# Autodesk Inventor assembly: TR1 Actuator
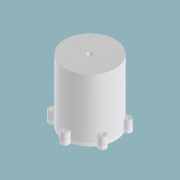
[picture p0: Inventor's stored thumbnail of the model, 180x180]
Saved by Autodesk Inventor 2017 SP1 (Build 210196100, 196)
## iProperties
Created: 2018-10-09
Part Number: TR1 Actuator
Document SubType Name: Assembly
Designer: Zach
Author: Zach
## Documents named in this file (9)
- C:\Users\Zach\Documents\GitHub\TR2\TR2 Actuator.iam
- C:\Users\Zach\Documents\GitHub\TR2\TA01.ipt
- C:\Users\Zach\Documents\GitHub\TR2\TA02.ipt
- C:\Users\Zach\Documents\GitHub\TR2\TR1 Actuator\Design Accelerator\Spur Gears2.iam
- C:\Users\Zach\Documents\GitHub\TR2\TR1 Actuator\Design Accelerator\Spur Gears3.iam
- C:\Users\Zach\Documents\GitHub\TR2\TA03.ipt
- C:\Users\Zach\Documents\GitHub\TR2\EMS22XXX-D28-LSX.ipt
- C:\Users\Zach\Documents\GitHub\TR2\12RPM Gear Motor.ipt
- C:\Users\Zach\Documents\GitHub\TR2\TR2 Arm.iam
## Components (11 placed, 7 different names)
1. TA01:1 — Mate:13, Mate:14, Mate:26
2. TA02:1 — Mate:2, Mate:3, Mate:4, Mate:5, Mate:6, Mate:7, Mate:8, Mate:14, Mate:16, Mate:17, Mate:18, Mate:19, Angle:1, Angle:2, Mate:20, Mate:21, Mate:22, Mate:24, Mate:25, Mate:26
3. Spur Gears:1 [sub-assembly] — Mate:2, Mate:25, Mate:27
4. Spur Gears:2 [sub-assembly] — Mate:3, Mate:4
5. Spur Gears:3 [sub-assembly] — Mate:5, Mate:6
6. TA03:1 — Mate:7, Mate:8, Mate:13, Mate:27
7. EMS22XXX-D28-LSX:1 — Mate:16, Mate:19, Angle:1, Mate:23
8. EMS22XXX-D28-LSX:2 — Mate:17, Mate:18, Angle:2
9. 12RPM Gear Motor:1 — Mate:20, Mate:21, Mate:22
10. Spur Gears:4 [sub-assembly] — Mate:23, Mate:24
11. TR2 Arm:1 [sub-assembly]
## Relationships (23: Mate 21, Angle 2)
- Mate:2: TA02:1 ↔ Spur Gears:1
- Mate:3: TA02:1 ↔ Spur Gears:2
- Mate:4: TA02:1 ↔ Spur Gears:2
- Mate:5: TA02:1 ↔ Spur Gears:3
- Mate:6: TA02:1 ↔ Spur Gears:3
- Mate:7: TA02:1 ↔ TA03:1
- Mate:8: TA02:1 ↔ TA03:1
- Mate:13: TA01:1 ↔ TA03:1
- Mate:14: TA01:1 ↔ TA02:1
- Mate:16: TA02:1 ↔ EMS22XXX-D28-LSX:1
- Mate:17: TA02:1 ↔ EMS22XXX-D28-LSX:2
- Mate:18: TA02:1 ↔ EMS22XXX-D28-LSX:2
- Mate:19: TA02:1 ↔ EMS22XXX-D28-LSX:1
- Angle:1 (0 deg): TA02:1 ↔ EMS22XXX-D28-LSX:1
- Angle:2 (0 deg): TA02:1 ↔ EMS22XXX-D28-LSX:2
- Mate:20: TA02:1 ↔ 12RPM Gear Motor:1
- Mate:21: TA02:1 ↔ 12RPM Gear Motor:1
- Mate:22: TA02:1 ↔ 12RPM Gear Motor:1
- Mate:23: EMS22XXX-D28-LSX:1 ↔ Spur Gears:4
- Mate:24: TA02:1 ↔ Spur Gears:4
- Mate:25: TA02:1 ↔ Spur Gears:1
- Mate:26: TA01:1 ↔ TA02:1
- Mate:27: Spur Gears:1 ↔ TA03:1
